# Autodesk Inventor assembly: DIN Block
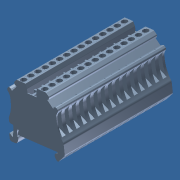
[picture p0: Inventor's stored thumbnail of the model, 180x180]
Saved by Autodesk Inventor 2012 (Build 160160000, 160)
## iProperties
Created: 2012-03-31
Part Number: DIN Block
Document SubType Name: Assembly
Designer: Edward
Author: Edward
## Documents named in this file (4)
- C:\Users\Edward\Documents\masters\CAD\DIN Terminal\DIN Block.iam
- C:\Users\Edward\Documents\masters\CAD\DIN Terminal\24v terminal.ipt
- C:\Users\Edward\Documents\masters\CAD\DIN Terminal\12v terminal.ipt
- C:\Users\Edward\Documents\masters\CAD\DIN Terminal\gnd terminal.ipt
## Components (15 placed, 3 different names)
1. 24v terminal:1 — Mate:2, Mate:3, Flush:12, Flush:13, Flush:26, Flush:27
2. 24v terminal:2 — Mate:3, Mate:4, Flush:11, Flush:12, Flush:25, Flush:26
3. 24v terminal:3 — Mate:1, Mate:2, Flush:13, Flush:14, Flush:27, Flush:28
4. 24v terminal:4 — Mate:1, Flush:14, Flush:28
5. 24v terminal:5 — Mate:14, Flush:1, Flush:15
6. 24v terminal:6 — Mate:13, Mate:14, Flush:1, Flush:2, Flush:15, Flush:16
7. 12v terminal:1 — Mate:12, Mate:13, Flush:2, Flush:3, Flush:16, Flush:17
8. 12v terminal:2 — Mate:11, Mate:12, Flush:3, Flush:4, Flush:17, Flush:18
9. 12v terminal:3 — Mate:10, Mate:11, Flush:4, Flush:5, Flush:18, Flush:19
10. gnd terminal:1 — Mate:9, Mate:10, Flush:5, Flush:6, Flush:19, Flush:20
11. gnd terminal:2 — Mate:8, Mate:9, Flush:6, Flush:7, Flush:20, Flush:21
12. gnd terminal:3 — Mate:7, Mate:8, Flush:7, Flush:8, Flush:21, Flush:22
13. gnd terminal:4 — Mate:5, Mate:6, Flush:9, Flush:10, Flush:23, Flush:24
14. gnd terminal:5 — Mate:4, Mate:5, Flush:10, Flush:11, Flush:24, Flush:25
15. gnd terminal:6 — Mate:6, Mate:7, Flush:8, Flush:9, Flush:22, Flush:23
## Relationships (42: Flush 28, Mate 14)
- Mate:1: 24v terminal:3 ↔ 24v terminal:4
- Mate:2: 24v terminal:1 ↔ 24v terminal:3
- Mate:3: 24v terminal:1 ↔ 24v terminal:2
- Mate:4: 24v terminal:2 ↔ gnd terminal:5
- Mate:5: gnd terminal:4 ↔ gnd terminal:5
- Mate:6: gnd terminal:4 ↔ gnd terminal:6
- Mate:7: gnd terminal:3 ↔ gnd terminal:6
- Mate:8: gnd terminal:2 ↔ gnd terminal:3
- Mate:9: gnd terminal:1 ↔ gnd terminal:2
- Mate:10: 12v terminal:3 ↔ gnd terminal:1
- Mate:11: 12v terminal:2 ↔ 12v terminal:3
- Mate:12: 12v terminal:1 ↔ 12v terminal:2
- Mate:13: 24v terminal:6 ↔ 12v terminal:1
- Mate:14: 24v terminal:5 ↔ 24v terminal:6
- Flush:1: 24v terminal:5 ↔ 24v terminal:6
- Flush:2: 24v terminal:6 ↔ 12v terminal:1
- Flush:3: 12v terminal:1 ↔ 12v terminal:2
- Flush:4: 12v terminal:2 ↔ 12v terminal:3
- Flush:5: 12v terminal:3 ↔ gnd terminal:1
- Flush:6: gnd terminal:1 ↔ gnd terminal:2
- Flush:7: gnd terminal:2 ↔ gnd terminal:3
- Flush:8: gnd terminal:3 ↔ gnd terminal:6
- Flush:9: gnd terminal:4 ↔ gnd terminal:6
- Flush:10: gnd terminal:4 ↔ gnd terminal:5
- Flush:11: 24v terminal:2 ↔ gnd terminal:5
- Flush:12: 24v terminal:1 ↔ 24v terminal:2
- Flush:13: 24v terminal:1 ↔ 24v terminal:3
- Flush:14: 24v terminal:3 ↔ 24v terminal:4
- Flush:15: 24v terminal:5 ↔ 24v terminal:6
- Flush:16: 24v terminal:6 ↔ 12v terminal:1
- Flush:17: 12v terminal:1 ↔ 12v terminal:2
- Flush:18: 12v terminal:2 ↔ 12v terminal:3
- Flush:19: 12v terminal:3 ↔ gnd terminal:1
- Flush:20: gnd terminal:1 ↔ gnd terminal:2
- Flush:21: gnd terminal:2 ↔ gnd terminal:3
- Flush:22: gnd terminal:3 ↔ gnd terminal:6
- Flush:23: gnd terminal:4 ↔ gnd terminal:6
- Flush:24: gnd terminal:4 ↔ gnd terminal:5
- Flush:25: 24v terminal:2 ↔ gnd terminal:5
- Flush:26: 24v terminal:1 ↔ 24v terminal:2
- Flush:27: 24v terminal:1 ↔ 24v terminal:3
- Flush:28: 24v terminal:3 ↔ 24v terminal:4
